# Autodesk Inventor assembly: analysis
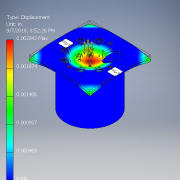
[picture p0: Inventor's stored thumbnail of the model, 180x180]
Saved by Autodesk Inventor 2018 (Build 220112000, 112)
## iProperties
Created: 2018-08-09
Part Number: analysis
Document SubType Name: Assembly
Designer: QITI
Author: QITI
## Documents named in this file (9)
- C:\Users\freyja\Documents\Cryorefrigerator\CAD\analysis.iam
- C:\Users\freyja\Documents\Cryorefrigerator\CAD\Top Plate.ipt
- C:\Users\freyja\Documents\Cryorefrigerator\CAD\vacuum jacket long.ipt
- C:\Users\freyja\Documents\Cryorefrigerator\CAD\analysis\AIP\FEA\cmlkwq6lc.fins
- C:\Users\freyja\Documents\Cryorefrigerator\CAD\analysis\AIP\FEA\cmlkwq6lc.fsat
- C:\Users\freyja\Documents\Cryorefrigerator\CAD\analysis\AIP\FEA\cmlkwq6lc.ftes
- C:\Users\freyja\Documents\Cryorefrigerator\CAD\analysis\AIP\FEA\cmlkwq6lc.fwiz
- C:\Users\freyja\Documents\Cryorefrigerator\CAD\analysis\AIP\FEA\cmlkwq6m8.fmsh
- C:\Users\freyja\Documents\Cryorefrigerator\CAD\analysis\AIP\FEA\cmlkzhy0w.fres
## Components (2 placed, 2 different names)
1. Top Plate:1 — Mate:4, Mate:5, Mate:6
2. vacuum jacket long:1 — Mate:4, Mate:5, Mate:6
## Relationships (3: Mate 3)
- Mate:4: Top Plate:1 ↔ vacuum jacket long:1
- Mate:5: Top Plate:1 ↔ vacuum jacket long:1
- Mate:6: Top Plate:1 ↔ vacuum jacket long:1
## Named parameters: sa_0 = 1034.21
note: some values were not read from the file. Shown as the stored number, unit unknown: "sa_0".
